# Autodesk Inventor assembly: Cuerpo-Rediseno-Ensamble
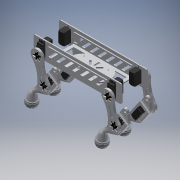
[picture p0: Inventor's stored thumbnail of the model, 180x180]
Saved by Autodesk Inventor 2019 (Build 230136000, 136)
## iProperties
Created: 2020-02-20
Part Number: Cuerpo-Rediseno-Ensamble
Document SubType Name: Assembly
Designer: jacqu
Author: jacqu
## Documents named in this file (8)
- E:\Escritorio\Temporal\Documentos\Robótica I\Robótica I - Proyecto Cuadrúpedo\Cuadrúpedo - Ensamble 2 DOF.iam
- E:\Escritorio\Temporal\Documentos\Robótica I\Robótica I - Proyecto Cuadrúpedo\Cuerpo - Base.ipt
- E:\Escritorio\Temporal\Documentos\Robótica I\Robótica I - Proyecto Cuadrúpedo\Cuerpo - Lateral.ipt
- E:\Escritorio\Temporal\Documentos\Robótica I\Robótica I - Proyecto Cuadrúpedo\Pata - Antebrazo.ipt
- E:\Escritorio\Temporal\Documentos\Robótica I\Robótica I - Proyecto Cuadrúpedo\Pata - Brazo - Pata Ninjaflex.ipt
- E:\Escritorio\Temporal\Documentos\Robótica I\Robótica I - Proyecto Cuadrúpedo\Servo MG996R\Servo MG996R - Ensamble - Sin Flor.iam
- E:\Escritorio\Temporal\Documentos\Robótica I\Robótica I - Proyecto Cuadrúpedo\Servo MG996R\TowerPro SG5010 - Acople Hélice.ipt
- E:\Escritorio\Temporal\Documentos\Robótica I\Robótica I - Proyecto Cuadrúpedo\Pata - Pie - Textura.ipt
## Components (31 placed, 7 different names)
1. Cuerpo - Base:1 — Mate:7, Mate:8, Mate:16
2. Cuerpo - Lateral:1 — Mate:7, Mate:8, Mate:16, Mate:17, Coincidencia:21, Coincidencia:22, Coincidencia:23, Coincidencia:27, Coincidencia:28, Coincidencia:29
3. Cuerpo - Lateral:2 — Mate:17, Coincidencia:18, Coincidencia:19, Coincidencia:20, Coincidencia:24, Coincidencia:25, Coincidencia:26
4. Servo MG996R - Ensamble - Sin Flor:1 [sub-assembly] — Coincidencia:18, Coincidencia:19, Coincidencia:20, Nivelación:8, Coincidencia:84
5. Servo MG996R - Ensamble - Sin Flor:2 [sub-assembly] — Coincidencia:24, Coincidencia:25, Coincidencia:26, Nivelación:5, Coincidencia:62
6. Servo MG996R - Ensamble - Sin Flor:3 [sub-assembly] — Coincidencia:21, Coincidencia:22, Coincidencia:23, Nivelación:2, Coincidencia:31, Coincidencia:54
7. Servo MG996R - Ensamble - Sin Flor:4 [sub-assembly] — Coincidencia:27, Coincidencia:28, Coincidencia:29, Nivelación:1, Coincidencia:30, Coincidencia:33
8. TowerPro SG5010 - Acople Hélice:1 — Nivelación:1, Coincidencia:30, Coincidencia:32, Coincidencia:34
9. TowerPro SG5010 - Acople Hélice:2 — Nivelación:2, Coincidencia:31, Coincidencia:53, Coincidencia:55
10. Pata - Antebrazo:1 — Coincidencia:32, Coincidencia:33, Coincidencia:34, Coincidencia:35, Coincidencia:36, Coincidencia:37
11. TowerPro SG5010 - Acople Hélice:3 — Coincidencia:35, Coincidencia:36, Coincidencia:37, Nivelación:3, Coincidencia:41
12. Pata - Brazo - Pata Ninjaflex:1 — Coincidencia:38, Coincidencia:39, Coincidencia:40, Coincidencia:42, Coincidencia:43
13. Servo MG996R - Ensamble - Sin Flor:5 [sub-assembly] — Coincidencia:38, Coincidencia:39, Coincidencia:40, Nivelación:3, Coincidencia:41
14. Pata - Pie - Textura:1 — Coincidencia:42, Coincidencia:43
15. Pata - Antebrazo:2 — Coincidencia:53, Coincidencia:54, Coincidencia:55
16. TowerPro SG5010 - Acople Hélice:4
17. Pata - Brazo - Pata Ninjaflex:2
18. Servo MG996R - Ensamble - Sin Flor:6 [sub-assembly]
19. Pata - Pie - Textura:2
20. Pata - Antebrazo:4 — Coincidencia:56, Coincidencia:57, Coincidencia:58, Coincidencia:59, Coincidencia:60, Coincidencia:61
21. TowerPro SG5010 - Acople Hélice:6 — Coincidencia:59, Coincidencia:60, Coincidencia:61, Nivelación:6, Coincidencia:71
22. TowerPro SG5010 - Acople Hélice:7 — Coincidencia:56, Coincidencia:57, Coincidencia:58, Nivelación:5, Coincidencia:62
23. Servo MG996R - Ensamble - Sin Flor:7 [sub-assembly] — Coincidencia:68, Coincidencia:69, Coincidencia:70, Nivelación:6, Coincidencia:71
24. Pata - Brazo - Pata Ninjaflex:3 — Coincidencia:68, Coincidencia:69, Coincidencia:70
25. Pata - Pie - Textura:3
26. Pata - Antebrazo:5
27. TowerPro SG5010 - Acople Hélice:8
28. TowerPro SG5010 - Acople Hélice:9 — Nivelación:8, Coincidencia:84
29. Servo MG996R - Ensamble - Sin Flor:8 [sub-assembly]
30. Pata - Brazo - Pata Ninjaflex:4
31. Pata - Pie - Textura:4
## Relationships (76: Mate 68, Flush 8)
- Mate:7: Cuerpo - Base:1 ↔ Cuerpo - Lateral:1
- Mate:8: Cuerpo - Base:1 ↔ Cuerpo - Lateral:1
- Mate:16 (-3.3 mm): Cuerpo - Base:1 ↔ Cuerpo - Lateral:1
- Mate:17 (83.3 mm): Cuerpo - Lateral:1 ↔ Cuerpo - Lateral:2
- Coincidencia:18 [Mate]: Cuerpo - Lateral:2 ↔ Servo MG996R - Ensamble - Sin Flor:1
- Coincidencia:19 [Mate]: Cuerpo - Lateral:2 ↔ Servo MG996R - Ensamble - Sin Flor:1
- Coincidencia:20 [Mate]: Cuerpo - Lateral:2 ↔ Servo MG996R - Ensamble - Sin Flor:1
- Coincidencia:21 [Mate]: Cuerpo - Lateral:1 ↔ Servo MG996R - Ensamble - Sin Flor:3
- Coincidencia:22 [Mate]: Cuerpo - Lateral:1 ↔ Servo MG996R - Ensamble - Sin Flor:3
- Coincidencia:23 [Mate]: Cuerpo - Lateral:1 ↔ Servo MG996R - Ensamble - Sin Flor:3
- Coincidencia:24 [Mate]: Cuerpo - Lateral:2 ↔ Servo MG996R - Ensamble - Sin Flor:2
- Coincidencia:25 [Mate]: Cuerpo - Lateral:2 ↔ Servo MG996R - Ensamble - Sin Flor:2
- Coincidencia:26 [Mate]: Cuerpo - Lateral:2 ↔ Servo MG996R - Ensamble - Sin Flor:2
- Coincidencia:27 [Mate]: Cuerpo - Lateral:1 ↔ Servo MG996R - Ensamble - Sin Flor:4
- Coincidencia:28 [Mate]: Cuerpo - Lateral:1 ↔ Servo MG996R - Ensamble - Sin Flor:4
- Coincidencia:29 [Mate]: Cuerpo - Lateral:1 ↔ Servo MG996R - Ensamble - Sin Flor:4
- Nivelación:1 [Flush]: Servo MG996R - Ensamble - Sin Flor:4 ↔ TowerPro SG5010 - Acople Hélice:1
- Coincidencia:30 [Mate]: Servo MG996R - Ensamble - Sin Flor:4 ↔ TowerPro SG5010 - Acople Hélice:1
- Nivelación:2 [Flush]: Servo MG996R - Ensamble - Sin Flor:3 ↔ TowerPro SG5010 - Acople Hélice:2
- Coincidencia:31 [Mate]: Servo MG996R - Ensamble - Sin Flor:3 ↔ TowerPro SG5010 - Acople Hélice:2
- Coincidencia:32 [Mate]: TowerPro SG5010 - Acople Hélice:1 ↔ Pata - Antebrazo:1
- Coincidencia:33 [Mate]: Servo MG996R - Ensamble - Sin Flor:4 ↔ Pata - Antebrazo:1
- Coincidencia:34 [Mate]: TowerPro SG5010 - Acople Hélice:1 ↔ Pata - Antebrazo:1
- Coincidencia:35 [Mate]: Pata - Antebrazo:1 ↔ TowerPro SG5010 - Acople Hélice:3
- Coincidencia:36 [Mate]: Pata - Antebrazo:1 ↔ TowerPro SG5010 - Acople Hélice:3
- Coincidencia:37 [Mate]: Pata - Antebrazo:1 ↔ TowerPro SG5010 - Acople Hélice:3
- Coincidencia:38 [Mate]: Pata - Brazo - Pata Ninjaflex:1 ↔ Servo MG996R - Ensamble - Sin Flor:5
- Coincidencia:39 [Mate]: Pata - Brazo - Pata Ninjaflex:1 ↔ Servo MG996R - Ensamble - Sin Flor:5
- Coincidencia:40 [Mate]: Pata - Brazo - Pata Ninjaflex:1 ↔ Servo MG996R - Ensamble - Sin Flor:5
- Nivelación:3 [Flush]: TowerPro SG5010 - Acople Hélice:3 ↔ Servo MG996R - Ensamble - Sin Flor:5
- Coincidencia:41 [Mate]: TowerPro SG5010 - Acople Hélice:3 ↔ Servo MG996R - Ensamble - Sin Flor:5
- Coincidencia:42 [Mate]: Pata - Brazo - Pata Ninjaflex:1 ↔ Pata - Pie - Textura:1
- Coincidencia:43 [Mate]: Pata - Brazo - Pata Ninjaflex:1 ↔ Pata - Pie - Textura:1
- [Mate]: Pata - Antebrazo:2 ↔ TowerPro SG5010 - Acople Hélice:4
- [Mate]: Pata - Antebrazo:2 ↔ TowerPro SG5010 - Acople Hélice:4
- [Mate]: Pata - Antebrazo:2 ↔ TowerPro SG5010 - Acople Hélice:4
- [Mate]: Pata - Brazo - Pata Ninjaflex:2 ↔ Servo MG996R - Ensamble - Sin Flor:6
- [Mate]: Pata - Brazo - Pata Ninjaflex:2 ↔ Servo MG996R - Ensamble - Sin Flor:6
- [Mate]: Pata - Brazo - Pata Ninjaflex:2 ↔ Servo MG996R - Ensamble - Sin Flor:6
- [Flush]: TowerPro SG5010 - Acople Hélice:4 ↔ Servo MG996R - Ensamble - Sin Flor:6
- [Mate]: TowerPro SG5010 - Acople Hélice:4 ↔ Servo MG996R - Ensamble - Sin Flor:6
- [Mate]: Pata - Brazo - Pata Ninjaflex:2 ↔ Pata - Pie - Textura:2
- [Mate]: Pata - Brazo - Pata Ninjaflex:2 ↔ Pata - Pie - Textura:2
- Coincidencia:53 [Mate]: TowerPro SG5010 - Acople Hélice:2 ↔ Pata - Antebrazo:2
- Coincidencia:54 [Mate]: Servo MG996R - Ensamble - Sin Flor:3 ↔ Pata - Antebrazo:2
- Coincidencia:55 [Mate]: TowerPro SG5010 - Acople Hélice:2 ↔ Pata - Antebrazo:2
- Coincidencia:56 [Mate]: Pata - Antebrazo:4 ↔ TowerPro SG5010 - Acople Hélice:7
- Coincidencia:57 [Mate]: Pata - Antebrazo:4 ↔ TowerPro SG5010 - Acople Hélice:7
- Coincidencia:58 [Mate]: Pata - Antebrazo:4 ↔ TowerPro SG5010 - Acople Hélice:7
- Coincidencia:59 [Mate]: Pata - Antebrazo:4 ↔ TowerPro SG5010 - Acople Hélice:6
- Coincidencia:60 [Mate]: Pata - Antebrazo:4 ↔ TowerPro SG5010 - Acople Hélice:6
- Coincidencia:61 [Mate]: Pata - Antebrazo:4 ↔ TowerPro SG5010 - Acople Hélice:6
- Nivelación:5 [Flush]: Servo MG996R - Ensamble - Sin Flor:2 ↔ TowerPro SG5010 - Acople Hélice:7
- Coincidencia:62 [Mate]: Servo MG996R - Ensamble - Sin Flor:2 ↔ TowerPro SG5010 - Acople Hélice:7
- [Mate]: Pata - Brazo - Pata Ninjaflex:3 ↔ Pata - Pie - Textura:3
- [Mate]: Pata - Brazo - Pata Ninjaflex:3 ↔ Pata - Pie - Textura:3
- Coincidencia:68 [Mate]: Servo MG996R - Ensamble - Sin Flor:7 ↔ Pata - Brazo - Pata Ninjaflex:3
- Coincidencia:69 [Mate]: Servo MG996R - Ensamble - Sin Flor:7 ↔ Pata - Brazo - Pata Ninjaflex:3
- Coincidencia:70 [Mate]: Servo MG996R - Ensamble - Sin Flor:7 ↔ Pata - Brazo - Pata Ninjaflex:3
- Nivelación:6 [Flush]: TowerPro SG5010 - Acople Hélice:6 ↔ Servo MG996R - Ensamble - Sin Flor:7
- Coincidencia:71 [Mate]: TowerPro SG5010 - Acople Hélice:6 ↔ Servo MG996R - Ensamble - Sin Flor:7
- [Mate]: Pata - Antebrazo:5 ↔ TowerPro SG5010 - Acople Hélice:9
- [Mate]: Pata - Antebrazo:5 ↔ TowerPro SG5010 - Acople Hélice:9
- [Mate]: Pata - Antebrazo:5 ↔ TowerPro SG5010 - Acople Hélice:9
- [Mate]: Pata - Antebrazo:5 ↔ TowerPro SG5010 - Acople Hélice:8
- [Mate]: Pata - Antebrazo:5 ↔ TowerPro SG5010 - Acople Hélice:8
- [Mate]: Pata - Antebrazo:5 ↔ TowerPro SG5010 - Acople Hélice:8
- [Mate]: Pata - Brazo - Pata Ninjaflex:4 ↔ Pata - Pie - Textura:4
- [Mate]: Pata - Brazo - Pata Ninjaflex:4 ↔ Pata - Pie - Textura:4
- [Mate]: Servo MG996R - Ensamble - Sin Flor:8 ↔ Pata - Brazo - Pata Ninjaflex:4
- [Mate]: Servo MG996R - Ensamble - Sin Flor:8 ↔ Pata - Brazo - Pata Ninjaflex:4
- [Mate]: Servo MG996R - Ensamble - Sin Flor:8 ↔ Pata - Brazo - Pata Ninjaflex:4
- [Flush]: TowerPro SG5010 - Acople Hélice:8 ↔ Servo MG996R - Ensamble - Sin Flor:8
- [Mate]: TowerPro SG5010 - Acople Hélice:8 ↔ Servo MG996R - Ensamble - Sin Flor:8
- Nivelación:8 [Flush]: Servo MG996R - Ensamble - Sin Flor:1 ↔ TowerPro SG5010 - Acople Hélice:9
- Coincidencia:84 [Mate]: Servo MG996R - Ensamble - Sin Flor:1 ↔ TowerPro SG5010 - Acople Hélice:9
## Named parameters: sa_0 = 2.05244, sa_1 = -444.817, sa_2 = -4.44822e-13, d64_d54 = 0 mm, d65_d55 = 0 mm, d66_d56 = 0 mm, d67_d57 = 0 mm, d68_d58 = 0 mm, d69_d59 = 0 mm, d70_d60 = 0 mm, d71_d61 = 0 mm, d72_d62 = 0 mm, d73_d63 = 0 mm, d98_d62 = 0 mm, d99_d63 = 0 mm, d105_d87 = 0 mm, d106_d88 = 0 mm, d107_d89 = 0 mm, d108_d90 = 0 mm, d109_d91 = 0 mm, d110_d92 = 0 mm, d111_d98_d62 = 0 mm, d112_d99_d63 = 0 mm, d113_d100 = 0 mm, d114_d101 = 0 mm, d115_d102 = 0 mm, d116_d103 = 0 mm, d117_d104 = 0 mm
note: some values were not read from the file. Shown as the stored number, unit unknown: "sa_0", "sa_1", "sa_2".
